# Autodesk Inventor assembly: C-AFBD22-35W
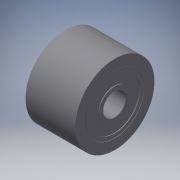
[picture p0: Inventor's stored thumbnail of the model, 180x180]
Saved by Autodesk Inventor 2019 (Build 230136000, 136)
## iProperties
Category: PARTsolutions
Company: MISUMI
Created: 2023-11-09
Part Number: C-AFBD22-35W
Catalog Web Link: www.cadenas.de
Description: C-AFBD, C-AFDF-Economy Idlers Backside Tension Type
Vendor: MISUMI
Document SubType Name: Assembly
Designer: psAdmin
Manufacturer: MISUMI
Mass: 17.0967 g
Surface Area: 89.6376 cm^2
Volume: 17.0967 cm^3
Density: 1 g/cm^3
Title: C-AFBD22-35W
Author: Cadenas PARTsolutions
Comments: Economy Idlers Backside Tension Type
PSOL_IDENT_0: {$CADENAS_DATA/23d-libs/misumi/metric/51_timing_pulleys/c_afbd_asmtab.prj},194 {VTYP=3D},{STYP=ASSTA
PSOL_IDENT_1: B},{NB=C-AFBD22-35W},{LINA=C-AFBD22-35W},{NN=C-AFBD, C-AFDF},{DATE=13.09.2022 06:49:12},{GEOMDATE=18
PSOL_IDENT_2: .05.2021 06:13:57},{VERSION=},{LINEID=100},{WBVAR=TS,TYPE},{WBNUMERIC=}  {NB=C-AFBD22-35W},{LINA=C-A
PSOL_IDENT_3: FBD22-35W},{KT=DUMMY},{PN=C-AFBD22-35W},{TS=BSB},{TSALG= 'CB','Center Bearing Type','BSB','Both Side
PSOL_IDENT_4: s Bearing Type' },{TYPE=C-AFBD},{TYPEALG= 'C-AFBD','No Flange','C-AFDF','Flanged' },{W=22.0},{NOM=35
PSOL_IDENT_5: W},{D=35},{F=45},{A=17.0},{ABI=-},{ABM=150},{S=0.00},{NO=6000ZZx2},{BN=6000},{DD=10},{B=8.0},{RR=-},
PSOL_IDENT_6: {E=30.000},{BD=26},{DH=23.000},{DD2=27.2},{RTT=1.200},{PTT=1.000},{CIF=0.000},{PPATH=c_afbd/c_afbd_a
PSOL_IDENT_7: smtpl.prj}
NB: C-AFBD22-35W
NN: C-AFBD, C-AFDF
NT: Economy Idlers Backside Tension Type
NBSYN: $PN.
LINA: C-AFBD22-35W
CATALOG: Misumi
PN: C-AFBD22-35W
TS: Both Sides Bearing Type
TYPE: No Flange
W: 22
NOM: 35W
D: 35
F: 45
A: 17
ABI: -
ABM: 150
S: 0
NO: 6000ZZx2
DD: 10
B: 8
RR: -
SUPPLIER: MISUMI
ARTICLENO: C-AFBD22-35W
BOMINFO: C-AFBD22-35W
CREATOR: CADENAS GmbH
## Documents named in this file (3)
- e:\temp\worker_COMMON_2\temp\tmp_7972_2_XniNt\format_0\C-AFBD22-35W.iam
- e:\temp\worker_COMMON_2\temp\tmp_7972_2_XniNt\format_0\C-AFBD22-35W_bw.ipt
- e:\temp\worker_COMMON_2\temp\tmp_7972_2_XniNt\format_0\bearing_6000.ipt
## Components (3 placed, 2 different names)
1. C-AFBD22-35W_bw:1 — b6000_1_XY@1 <-> center_point_XY@2, b6000_1_Z@1 <-> center_point_Z@2, b6000_1_YZ@1 <-> center_point_YZ@2, b6000_2_XY@1 <-> center_point_XY@3, b6000_2_Z@1 <-> center_point_Z@3, b6000_2_YZ@1 <-> center_point_YZ@3
2. bearing_6000:1 — b6000_1_XY@1 <-> center_point_XY@2, b6000_1_Z@1 <-> center_point_Z@2, b6000_1_YZ@1 <-> center_point_YZ@2
3. bearing_6000:2 — b6000_2_XY@1 <-> center_point_XY@3, b6000_2_Z@1 <-> center_point_Z@3, b6000_2_YZ@1 <-> center_point_YZ@3
## Relationships (6: Mate 4, Angle 2)
- b6000_1_XY@1 <-> center_point_XY@2 [Mate]: C-AFBD22-35W_bw:1 ↔ bearing_6000:1
- b6000_1_Z@1 <-> center_point_Z@2 [Mate]: C-AFBD22-35W_bw:1 ↔ bearing_6000:1
- b6000_1_YZ@1 <-> center_point_YZ@2 [Angle] (0 deg): C-AFBD22-35W_bw:1 ↔ bearing_6000:1
- b6000_2_XY@1 <-> center_point_XY@3 [Mate]: C-AFBD22-35W_bw:1 ↔ bearing_6000:2
- b6000_2_Z@1 <-> center_point_Z@3 [Mate]: C-AFBD22-35W_bw:1 ↔ bearing_6000:2
- b6000_2_YZ@1 <-> center_point_YZ@3 [Angle] (0 deg): C-AFBD22-35W_bw:1 ↔ bearing_6000:2
